# Autodesk Inventor assembly: yotukiude
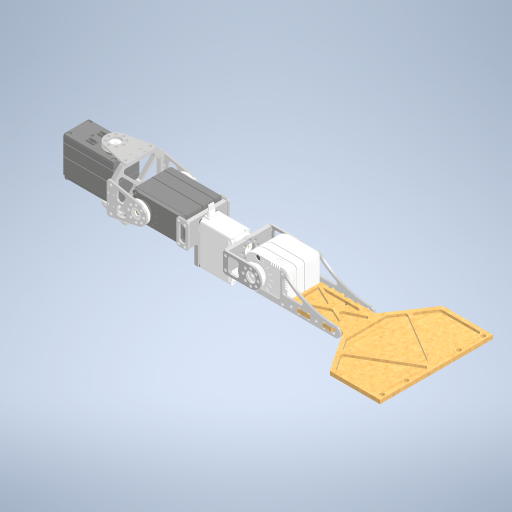
[picture p0: Inventor's stored thumbnail of the model, 512x512]
Saved by Autodesk Inventor 2024 (Build 280153000, 153)
## iProperties
Created: 2024-01-14
Part Number: yotukiude
Document SubType Name: Assembly
Designer: right
Author: right
## Documents named in this file (14)
- C:\Users\right\OneDrive\ドキュメント\Inventor\V2二足Light＿仮\yotukiude.iam
- C:\Users\right\OneDrive\ドキュメント\Inventor\V2二足Light＿仮\KRS2500_scale3.ipt
- C:\Users\right\OneDrive\ドキュメント\Inventor\V2二足Light＿仮\02159_SmallFreeHornC_MIR2.ipt
- C:\Users\right\OneDrive\ドキュメント\Inventor\V2二足Light＿仮\02157_SmallDiameterHornB_MIR1.ipt
- C:\Users\right\OneDrive\ドキュメント\Inventor\V2二足Light＿仮\kata_new.ipt
- C:\Users\right\OneDrive\ドキュメント\Inventor\V2二足Light＿仮\new_kata_3.ipt
- C:\Users\right\OneDrive\ドキュメント\Inventor\V2二足Light＿仮\kata_new_1.5.ipt
- C:\Users\right\OneDrive\ドキュメント\Inventor\V2二足Light＿仮\tesaki_arata.iam
- C:\Users\right\OneDrive\ドキュメント\Inventor\V2二足Light＿仮\hera_porika2.ipt
- C:\Users\right\OneDrive\ドキュメント\Inventor\V2二足Light＿仮\newnewude.ipt
- C:\Users\right\OneDrive\ドキュメント\Inventor\V2二足Light＿仮\udeyo.ipt
- C:\Users\right\OneDrive\ドキュメント\Inventor\V2二足Light＿仮\KRS3200_scale\KRS3200_scale.ipt
- C:\Users\right\OneDrive\ドキュメント\Inventor\V2二足Light＿仮\udeyi.ipt
- C:\Users\right\OneDrive\ドキュメント\Inventor\V2二足Light＿仮\tunage.ipt
## Components (23 placed, 13 different names)
1. KRS2500_scale3:1
2. 02159_SmallFreeHornC_MIR2:1
3. 02157_SmallDiameterHornB_MIR1:1
4. kata_new:1
5. new_kata_3:1 — 角度:4
6. kata_new:2
7. kata_new_1.5:1
8. kata_new_1.5:2
9. KRS2500_scale3:2 — 挿入:33, 挿入:34
10. 02159_SmallFreeHornC_MIR2:2
11. 02157_SmallDiameterHornB_MIR1:2
12. 02159_SmallFreeHornC_MIR2:3 — 挿入:50, 挿入:51
13. tesaki_arata:1 [sub-assembly] — 挿入:52, 角度:3
14. hera_porika2:1 — 角度:2, 挿入:52
15. 02157_SmallDiameterHornB_MIR1:3 — 挿入:44, 挿入:45
16. newnewude:1 — 挿入:37, 挿入:38
17. newnewude:2 — 挿入:33, 挿入:34, 挿入:35, 挿入:36, 角度:3
18. udeyo:1 — 挿入:35, 挿入:36, 挿入:37, 挿入:38, 挿入:39, 挿入:40
19. KRS3200_scale:1 — 挿入:39, 挿入:40, 挿入:41, 角度:2, 角度:4
20. 02157_SmallDiameterHornB_MIR1:4 — 挿入:41, 挿入:42, 挿入:43
21. udeyi:1 — 挿入:42, 挿入:43, 挿入:46, 挿入:47, 挿入:48, 挿入:49
22. tunage:1 — 挿入:44, 挿入:45, 挿入:46, 挿入:47
23. tunage:2 — 挿入:48, 挿入:49, 挿入:50, 挿入:51
## Relationships (50: Insert 44, Angle 4, Flush 2)
- [Insert]: KRS2500_scale3:1 ↔ 02159_SmallFreeHornC_MIR2:1
- [Insert]: KRS2500_scale3:1 ↔ 02157_SmallDiameterHornB_MIR1:1
- [Flush]: 02157_SmallDiameterHornB_MIR1:1 ↔ kata_new:1
- [Insert]: 02157_SmallDiameterHornB_MIR1:1 ↔ kata_new:1
- [Insert]: 02157_SmallDiameterHornB_MIR1:1 ↔ kata_new:1
- [Flush]: kata_new:1 ↔ new_kata_3:1
- [Insert]: 02159_SmallFreeHornC_MIR2:1 ↔ kata_new:2
- [Insert]: 02159_SmallFreeHornC_MIR2:1 ↔ kata_new:2
- [Insert]: new_kata_3:1 ↔ kata_new:2
- [Insert]: kata_new:1 ↔ new_kata_3:1
- [Insert]: kata_new:1 ↔ new_kata_3:1
- [Insert]: new_kata_3:1 ↔ kata_new:2
- [Insert]: new_kata_3:1 ↔ kata_new_1.5:1
- [Insert]: new_kata_3:1 ↔ kata_new_1.5:1
- [Insert]: new_kata_3:1 ↔ kata_new_1.5:2
- [Insert]: new_kata_3:1 ↔ kata_new_1.5:2
- [Insert]: KRS2500_scale3:2 ↔ 02159_SmallFreeHornC_MIR2:2
- [Insert]: KRS2500_scale3:2 ↔ 02157_SmallDiameterHornB_MIR1:2
- [Insert]: kata_new_1.5:1 ↔ 02157_SmallDiameterHornB_MIR1:2
- [Insert]: kata_new_1.5:1 ↔ 02157_SmallDiameterHornB_MIR1:2
- [Insert]: kata_new_1.5:2 ↔ 02159_SmallFreeHornC_MIR2:2
- [Insert]: kata_new_1.5:2 ↔ 02159_SmallFreeHornC_MIR2:2
- [Angle] (0 deg): KRS2500_scale3:1 ↔ new_kata_3:1
- [Insert]: tesaki_arata:1 ↔ hera_porika2:1
- [Insert]: tesaki_arata:1 ↔ 02157_SmallDiameterHornB_MIR1:3
- [Insert]: KRS2500_scale3:2 ↔ newnewude:1
- [Insert]: 02159_SmallFreeHornC_MIR2:3 ↔ tesaki_arata:1
- 挿入:33 [Insert]: KRS2500_scale3:2 ↔ newnewude:2
- 挿入:34 [Insert]: KRS2500_scale3:2 ↔ newnewude:2
- 挿入:35 [Insert]: newnewude:2 ↔ udeyo:1
- 挿入:36 [Insert]: newnewude:2 ↔ udeyo:1
- 挿入:37 [Insert]: newnewude:1 ↔ udeyo:1
- 挿入:38 [Insert]: newnewude:1 ↔ udeyo:1
- 挿入:39 [Insert]: udeyo:1 ↔ KRS3200_scale:1
- 挿入:40 [Insert]: udeyo:1 ↔ KRS3200_scale:1
- 挿入:41 [Insert]: KRS3200_scale:1 ↔ 02157_SmallDiameterHornB_MIR1:4
- 挿入:42 [Insert]: 02157_SmallDiameterHornB_MIR1:4 ↔ udeyi:1
- 挿入:43 [Insert]: 02157_SmallDiameterHornB_MIR1:4 ↔ udeyi:1
- 挿入:44 [Insert]: 02157_SmallDiameterHornB_MIR1:3 ↔ tunage:1
- 挿入:45 [Insert]: 02157_SmallDiameterHornB_MIR1:3 ↔ tunage:1
- 挿入:46 [Insert]: udeyi:1 ↔ tunage:1
- 挿入:47 [Insert]: udeyi:1 ↔ tunage:1
- 挿入:48 [Insert]: udeyi:1 ↔ tunage:2
- 挿入:49 [Insert]: udeyi:1 ↔ tunage:2
- 挿入:50 [Insert]: 02159_SmallFreeHornC_MIR2:3 ↔ tunage:2
- 挿入:51 [Insert]: 02159_SmallFreeHornC_MIR2:3 ↔ tunage:2
- 角度:2 [Angle] (0 deg): hera_porika2:1 ↔ KRS3200_scale:1
- 挿入:52 [Insert]: tesaki_arata:1 ↔ hera_porika2:1
- 角度:3 [Angle] (0 deg): tesaki_arata:1 ↔ newnewude:2
- 角度:4 [Angle] (0 deg): new_kata_3:1 ↔ KRS3200_scale:1
## Named parameters: d20_d1 = 0 mm, d21_d0 = 0 mm, d6_d22 = 0 mm, d6_d23 = 0 mm, d7_d25 = 0 mm, d8_d26 = 0 mm, d22_d29 = 0 deg
